# Autodesk Inventor assembly: Assembly3D_print
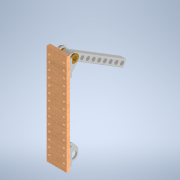
[picture p0: Inventor's stored thumbnail of the model, 180x180]
Saved by Autodesk Inventor 2022 (Build 260153000, 153)
## iProperties
Created: 2022-04-10
Part Number: Assembly3D_print
Document SubType Name: Assembly
Designer: Patrick
Author: Patrick
## Documents named in this file (5)
- H:\OneDrive - Syddansk Universitet\2. Semester Master\Mekaniske Elementer\Mini Project\2020-10-23\Workspaces\Workspace\Assembly3D_print.iam
- H:\OneDrive - Syddansk Universitet\2. Semester Master\Mekaniske Elementer\Mini Project\2020-10-23\Workspaces\Workspace\board.ipt
- H:\OneDrive - Syddansk Universitet\2. Semester Master\Mekaniske Elementer\Mini Project\2020-10-23\Workspaces\Workspace\beslag_board_3D.ipt
- H:\OneDrive - Syddansk Universitet\2. Semester Master\Mekaniske Elementer\Mini Project\2020-10-23\Workspaces\Workspace\Stang3D.ipt
- H:\OneDrive - Syddansk Universitet\2. Semester Master\Mekaniske Elementer\Mini Project\2020-10-23\Workspaces\Workspace\bøsning_beslag_3D.ipt
## Components (6 placed, 4 different names)
1. board:1 — Rigid:1, Rigid:2
2. beslag_board_3D:1 — Rigid:1, Rotational:1, Rotational:2, Rotational:3
3. beslag_board_3D:2 — Rigid:2
4. Stang3D:1 — Rotational:1
5. bøsning_beslag_3D:1 — Rotational:2
6. bøsning_beslag_3D:2 — Rotational:3
## Relationships (5: RevoluteJoint 3, WeldJoint 2)
- Rigid:1 [WeldJoint]: board:1 ↔ beslag_board_3D:1
- Rigid:2 [WeldJoint]: board:1 ↔ beslag_board_3D:2
- Rotational:1 [RevoluteJoint]: beslag_board_3D:1 ↔ Stang3D:1
- Rotational:2 [RevoluteJoint]: beslag_board_3D:1 ↔ bøsning_beslag_3D:1
- Rotational:3 [RevoluteJoint]: beslag_board_3D:1 ↔ bøsning_beslag_3D:2
